# Autodesk Inventor assembly: WheelAssembly
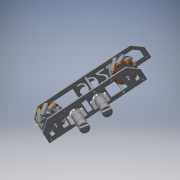
[picture p0: Inventor's stored thumbnail of the model, 180x180]
Saved by Autodesk Inventor 2017 (Build 210142000, 142)
## iProperties
Created: 2016-09-10
Part Number: WheelAssembly
Document SubType Name: Assembly
Designer: RoboticsUser
Author: RoboticsUser
## Documents named in this file (13)
- C:\Robotics\CAD\2016-17_CAD\DriveTrain\WheelAssemble2.0-right.iam
- C:\Robotics\CAD\COTSParts\Actobotics\545 parts\545556.ipt
- C:\Robotics\CAD\COTSParts\Actobotics\615 parts\615102.ipt
- C:\Robotics\CAD\COTSParts\Actobotics\634 parts\634080.ipt
- C:\Robotics\CAD\COTSParts\Motors\Andymark 2964  NeveRest 40 Motor.ipt
- C:\Robotics\CAD\COTSParts\Tetrix\tetrix-motor-mounts-1.snapshot.1\Tetrex 2pc motor mount.ipt
- C:\Robotics\CAD\COTSParts\Actobotics\545 parts\545456.ipt
- C:\Robotics\CAD\COTSParts\Wheels\AndyMark Mecanum Wheels\100mm Aluminum Mecanum wheels.ipt
- C:\Robotics\CAD\2016-17_CAD\DriveTrain\DriveTrainPlate2.0RightOutside.iam
- C:\Robotics\CAD\2016-17_CAD\DriveTrain\DriveTrainPlate2.0RightInside.ipt
- C:\Robotics\CAD\COTSParts\Actobotics\535 parts\535198.ipt
- C:\Robotics\CAD\COTSParts\Actobotics\collar.ipt
- C:\Robotics\CAD\2016-17_CAD\DriveTrain\drive train standoff.ipt
## Components (35 placed, 12 different names)
1. 545556:2 — Mate:73, Mate:74, Mate:75, Mate:76, Mate:77
2. 615102:4 — Mate:36, Mate:37, Mate:84
3. 634080:2 — Mate:77, Mate:79, Mate:81, Mate:89, Mate:90, Mate:93, Mate:94, Insert:113, Flush:3
4. 545556:6 — Insert:83, Mate:46
5. 615102:5 — Mate:44, Mate:46, Mate:118
6. 634080:3 — Mate:28, Mate:30, Mate:44, Mate:50, Mate:91, Mate:92, Mate:95, Mate:113, Mate:114, Mate:116, Flush:2
7. Andymark 2964  NeveRest 40 Motor:2 — Insert:105, Mate:111, Mate:127
8. 545556:8 — Insert:112
9. 545556:9 — Mate:37, Mate:38
10. Andymark 2964  NeveRest 40 Motor:3 — Mate:36, Mate:38, Mate:71, Flush:1, Mate:84
11. Tetrex 2pc motor mount:1 — Mate:109, Mate:127, Mate:128
12. Tetrex 2pc motor mount:2 — Mate:107, Mate:108, Mate:126
13. 545456:1 — Mate:75, Mate:76, Mate:80
14. 545456:3 — Insert:83, Insert:88
15. 615102:6 — Mate:111, Mate:112, Insert:112
16. 615102:7 — Mate:73, Mate:74
17. 100mm Aluminum Mecanum wheels:1 — Insert:88, Mate:27, Mate:50
18. 100mm Aluminum Mecanum wheels:2 — Mate:79, Mate:80, Mate:82
19. 545456:4 — Insert:106, Mate:82
20. 545456:5 — Mate:27, Mate:28, Mate:121
21. 545556:12 — Mate:30, Mate:119, Mate:121
22. 545556:13 — Insert:106, Mate:81, Mate:120
23. DriveTrainPlate2.0RightOutside:1 [sub-assembly] — Insert:108, Mate:113, Mate:117, Mate:119, Mate:120, Mate:122, Mate:123, Mate:130, Mate:131, Mate:133, Flush:4, Flush:5
24. DriveTrainPlate2.0RightInside:1 — Insert:105, Mate:71, Flush:1, Insert:109, Mate:107, Mate:108, Mate:109, Mate:112, Mate:114, Mate:118, Mate:124, Mate:125, Mate:126, Mate:128, Mate:129, Mate:132, Mate:134, Flush:4, Flush:5
25. 535198:1 — Mate:90, Insert:109
26. 535198:2 — Mate:116, Mate:117
27. 535198:3 — Mate:89, Insert:108
28. 535198:4 — Mate:91
29. collar:1 — Mate:94, Insert:113, Mate:122, Flush:3
30. collar:2 — Mate:95, Mate:123, Flush:2
31. collar:3 — Mate:92, Mate:124
32. collar:4 — Mate:93, Mate:125
33. drive train standoff:1 — Mate:133, Mate:134
34. drive train standoff:2 — Mate:129, Mate:130
35. drive train standoff:3 — Mate:131, Mate:132
## Relationships (66: Mate 53, Insert 8, Flush 5)
- Insert:83: 545556:6 ↔ 545456:3
- Insert:88: 545456:3 ↔ 100mm Aluminum Mecanum wheels:1
- Mate:27: 100mm Aluminum Mecanum wheels:1 ↔ 545456:5
- Mate:28: 634080:3 ↔ 545456:5
- Mate:30: 634080:3 ↔ 545556:12
- Mate:36: 615102:4 ↔ Andymark 2964  NeveRest 40 Motor:3
- Mate:37: 615102:4 ↔ 545556:9
- Mate:38: 545556:9 ↔ Andymark 2964  NeveRest 40 Motor:3
- Mate:44: 615102:5 ↔ 634080:3
- Mate:46: 545556:6 ↔ 615102:5
- Mate:50: 634080:3 ↔ 100mm Aluminum Mecanum wheels:1
- Insert:105: Andymark 2964  NeveRest 40 Motor:2 ↔ DriveTrainPlate2.0RightInside:1
- Mate:71: Andymark 2964  NeveRest 40 Motor:3 ↔ DriveTrainPlate2.0RightInside:1
- Flush:1: Andymark 2964  NeveRest 40 Motor:3 ↔ DriveTrainPlate2.0RightInside:1
- Mate:73: 545556:2 ↔ 615102:7
- Mate:74: 545556:2 ↔ 615102:7
- Mate:75: 545556:2 ↔ 545456:1
- Mate:76: 545556:2 ↔ 545456:1
- Mate:77: 545556:2 ↔ 634080:2
- Mate:79: 634080:2 ↔ 100mm Aluminum Mecanum wheels:2
- Mate:80: 545456:1 ↔ 100mm Aluminum Mecanum wheels:2
- Insert:106: 545456:4 ↔ 545556:13
- Mate:81: 634080:2 ↔ 545556:13
- Mate:82: 100mm Aluminum Mecanum wheels:2 ↔ 545456:4
- Mate:84 (6.35 mm): 615102:4 ↔ Andymark 2964  NeveRest 40 Motor:3
- Mate:89: 634080:2 ↔ 535198:3
- Mate:90: 634080:2 ↔ 535198:1
- Mate:91: 634080:3 ↔ 535198:4
- Insert:108: DriveTrainPlate2.0RightOutside:1 ↔ 535198:3
- Insert:109: DriveTrainPlate2.0RightInside:1 ↔ 535198:1
- Mate:92: 634080:3 ↔ collar:3
- Mate:93: 634080:2 ↔ collar:4
- Mate:94: 634080:2 ↔ collar:1
- Mate:95: 634080:3 ↔ collar:2
- Mate:107: Tetrex 2pc motor mount:2 ↔ DriveTrainPlate2.0RightInside:1
- Mate:108: Tetrex 2pc motor mount:2 ↔ DriveTrainPlate2.0RightInside:1
- Mate:109: Tetrex 2pc motor mount:1 ↔ DriveTrainPlate2.0RightInside:1
- Mate:111: Andymark 2964  NeveRest 40 Motor:2 ↔ 615102:6
- Mate:112 (6.35 mm): 615102:6 ↔ DriveTrainPlate2.0RightInside:1
- Insert:112 (-2.54 mm): 545556:8 ↔ 615102:6
- Insert:113: 634080:2 ↔ collar:1
- Mate:113: 634080:3 ↔ DriveTrainPlate2.0RightOutside:1
- Mate:114: 634080:3 ↔ DriveTrainPlate2.0RightInside:1
- Mate:116: 634080:3 ↔ 535198:2
- Mate:117: DriveTrainPlate2.0RightOutside:1 ↔ 535198:2
- Mate:118 (6.35 mm): 615102:5 ↔ DriveTrainPlate2.0RightInside:1
- Mate:119 (3.175 mm): 545556:12 ↔ DriveTrainPlate2.0RightOutside:1
- Mate:120 (3.175 mm): 545556:13 ↔ DriveTrainPlate2.0RightOutside:1
- Mate:121: 545456:5 ↔ 545556:12
- Mate:122: DriveTrainPlate2.0RightOutside:1 ↔ collar:1
- Mate:123: DriveTrainPlate2.0RightOutside:1 ↔ collar:2
- Mate:124: DriveTrainPlate2.0RightInside:1 ↔ collar:3
- Mate:125: DriveTrainPlate2.0RightInside:1 ↔ collar:4
- Flush:2: 634080:3 ↔ collar:2
- Flush:3: 634080:2 ↔ collar:1
- Mate:126: Tetrex 2pc motor mount:2 ↔ DriveTrainPlate2.0RightInside:1
- Mate:127: Andymark 2964  NeveRest 40 Motor:2 ↔ Tetrex 2pc motor mount:1
- Mate:128: Tetrex 2pc motor mount:1 ↔ DriveTrainPlate2.0RightInside:1
- Mate:129: DriveTrainPlate2.0RightInside:1 ↔ drive train standoff:2
- Mate:130: DriveTrainPlate2.0RightOutside:1 ↔ drive train standoff:2
- Mate:131: DriveTrainPlate2.0RightOutside:1 ↔ drive train standoff:3
- Mate:132: DriveTrainPlate2.0RightInside:1 ↔ drive train standoff:3
- Mate:133: DriveTrainPlate2.0RightOutside:1 ↔ drive train standoff:1
- Mate:134: DriveTrainPlate2.0RightInside:1 ↔ drive train standoff:1
- Flush:4: DriveTrainPlate2.0RightOutside:1 ↔ DriveTrainPlate2.0RightInside:1
- Flush:5: DriveTrainPlate2.0RightOutside:1 ↔ DriveTrainPlate2.0RightInside:1
